# Autodesk Inventor assembly: s-assy-pillar1
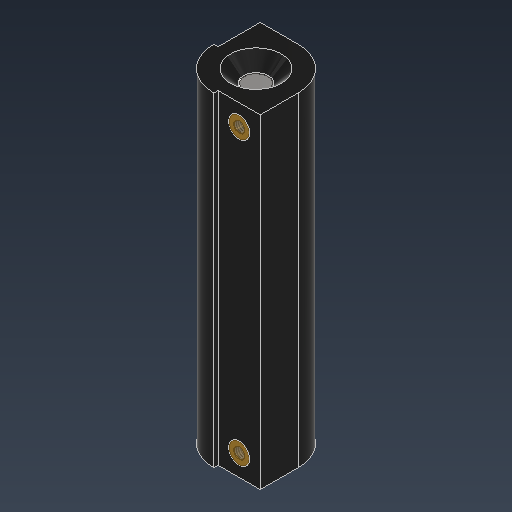
[picture p0: Inventor's stored thumbnail of the model, 512x512]
Saved by Autodesk Inventor 2021 (Build 250183000, 183)
## iProperties
Created: 2021-08-04
Part Number: s-assy-pillar1
Document SubType Name: Assembly
Designer: yuta0
Author: yuta0
## Documents named in this file (4)
- C:\Users\yuta0\Documents\GitHub\catchrobo_hardware\assy-robot\s-assy-pillar1.iam
- C:\Users\yuta0\Documents\GitHub\catchrobo_hardware\assy-robot\base4.ipt
- C:\Users\yuta0\Documents\GitHub\catchrobo_hardware\assy-robot\SB-305060.ipt
- C:\Users\yuta0\Documents\GitHub\catchrobo_hardware\assy-robot\holder_magnet.ipt
## Components (7 placed, 3 different names)
1. base4:1 — メイト:3, メイト:4, メイト:6, メイト:7, メイト:9, メイト:10, メイト:11, メイト:12
2. SB-305060:5 — メイト:9, メイト:10
3. holder_magnet:1 — メイト:11, メイト:12
4. SB-305060:2 — メイト:3, メイト:4
5. SB-305060:3 — メイト:6, メイト:7
6. SB-305060:6
7. SB-305060:7
## Component patterns: (2 elements, first: SB-305060:2 + SB-305060:3)
## Relationships (8: Mate 8)
- メイト:3 [Mate]: base4:1 ↔ SB-305060:2
- メイト:4 [Mate]: base4:1 ↔ SB-305060:2
- メイト:6 [Mate]: base4:1 ↔ SB-305060:3
- メイト:7 [Mate]: base4:1 ↔ SB-305060:3
- メイト:9 [Mate]: base4:1 ↔ SB-305060:5
- メイト:10 [Mate]: base4:1 ↔ SB-305060:5
- メイト:11 [Mate]: base4:1 ↔ holder_magnet:1
- メイト:12 [Mate]: base4:1 ↔ holder_magnet:1
